# Autodesk Inventor assembly: 6P Sprocket
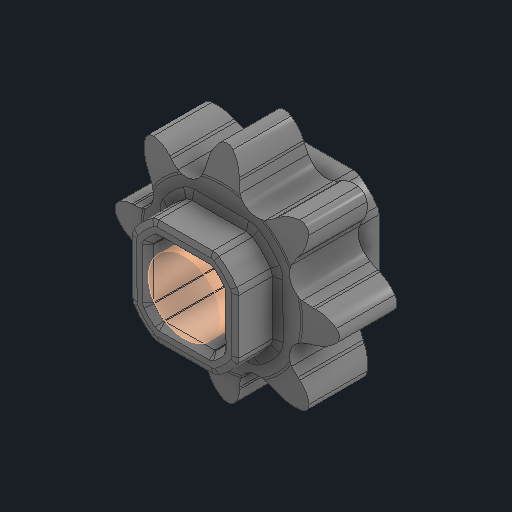
[picture p0: Inventor's stored thumbnail of the model, 512x512]
Saved by Autodesk Inventor 2025 (Build 290162000, 162)
## iProperties
Created: 2022-08-02
Part Number: 6P Sprocket
Document SubType Name: Assembly
Designer: ylu12
Author: ylu12
## Documents named in this file (3)
- D:\vex_robotics_high_stakes\hardware\cad\robpros_cad_lib\Motion\Sprockets\6P Sprocket\6P 8T Sprocket, No Insert.iam
- D:\vex_robotics_high_stakes\hardware\cad\robpros_cad_lib\Motion\Sprockets\Reference Files\6P 8T Sprocket.ipt
- D:\vex_robotics_high_stakes\hardware\cad\robpros_cad_lib\Motion\Sprockets\6P Sprocket.iam
## Components (1 placed, 1 different names)
1. 8T — Mate:5, Mate:6, Flush:3
## Relationships (3: Mate 2, Flush 1)
- Mate:5: 8T
- Mate:6: 8T
- Flush:3: 8T
